# Autodesk Inventor assembly: CompactSlide
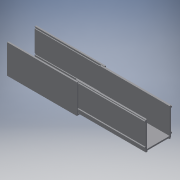
[picture p0: Inventor's stored thumbnail of the model, 180x180]
Saved by Autodesk Inventor 2017 (Build 210142000, 142)
## iProperties
Created: 2017-11-11
Part Number: CompactSlide
Document SubType Name: Assembly
Designer: User
Author: User
## Documents named in this file (3)
- C:\Robotics\CAD\2017-18_CAD\Prototypes\CompactSlide.iam
- C:\Robotics\CAD\2017-18_CAD\Prototypes\CompactSlidePart1.ipt
- C:\Robotics\CAD\2017-18_CAD\Prototypes\CompactSlidePart2.ipt
## Components (2 placed, 2 different names)
1. CompactSlidePart1:1 — Mate:1, Mate:2, Mate:3
2. CompactSlidePart2:1 — Mate:1, Mate:2, Mate:3
## Relationships (3: Mate 3)
- Mate:1: CompactSlidePart1:1 ↔ CompactSlidePart2:1
- Mate:2: CompactSlidePart1:1 ↔ CompactSlidePart2:1
- Mate:3 (-12.7 mm): CompactSlidePart1:1 ↔ CompactSlidePart2:1
